# Autodesk Inventor assembly: 细轴四方轴套用的螺丝螺帽套
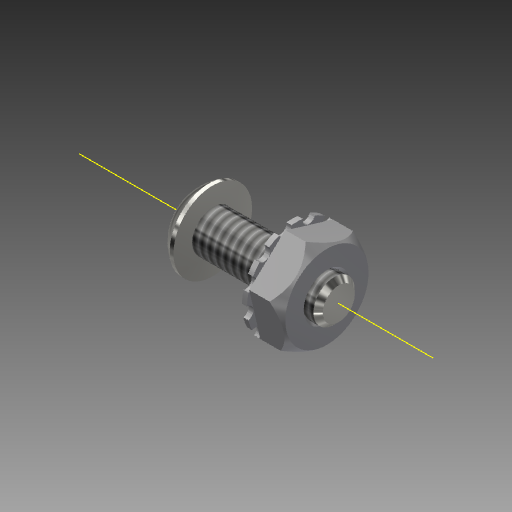
[picture p0: Inventor's stored thumbnail of the model, 512x512]
Saved by Autodesk Inventor 2019.4 (Build 234330000, 330)
## iProperties
Created: 2019-05-20
Part Number: 细轴四方轴套用的螺丝螺帽套
Material: 常规
Document SubType Name: Assembly
Designer: aresp
Author: aresp
## Documents named in this file (3)
- D:\2019-2020TowerTakeOverCad\ncrCadLib\细轴四方轴套用的螺丝螺帽套.iam
- D:\2019-2020TowerTakeOverCad\ncrCadLib\螺丝螺帽\Screw 8-32 x 0.500'' 三号.ipt
- D:\2019-2020TowerTakeOverCad\ncrCadLib\螺丝螺帽\普通螺帽.ipt
## Components (2 placed, 2 different names)
1. Screw 8-32 x 0.500'' 三号:1 — 配合:2
2. 普通螺帽:1 — 配合:2
## Relationships (2: Mate 2)
- [Mate]: Screw 8-32 x 0.500'' 三号:1 ↔ 普通螺帽:1
- 配合:2 [Mate] (7.925 mm): Screw 8-32 x 0.500'' 三号:1 ↔ 普通螺帽:1
